# Autodesk Inventor assembly: MG-Encoderplatine
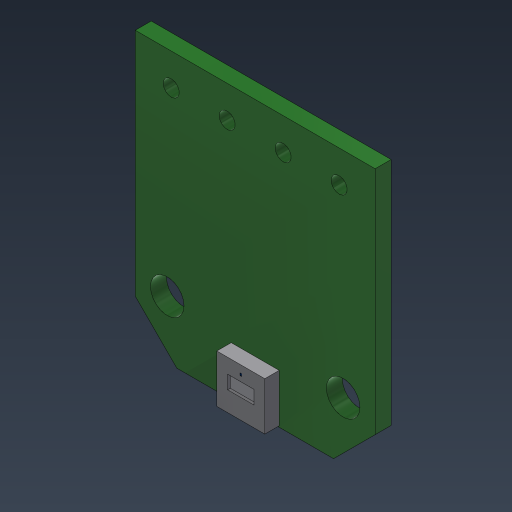
[picture p0: Inventor's stored thumbnail of the model, 512x512]
Saved by Autodesk Inventor 2023.1 (Build 271208000, 208)
## iProperties
Part Number: MG-Encoderplatine
Material: Generisch
Document SubType Name: Assembly
Designer: rYan
Mass: 0.362061 g
Surface Area: 6.73753 cm^2
Volume: 0.271556 cm^3
Density: 1.33328 g/cm^3
Author: rYan
## Documents named in this file (3)
- D:\TIGERsGIT\Hardware\mechanik\2024\Inventor\Robot\Drive Train\Common\MG-Encoderplatine.iam
- D:\TIGERsGIT\Hardware\mechanik\2024\Inventor\Robot\Drive Train\Common\Encoderplatine.ipt
- D:\TIGERsGIT\Hardware\mechanik\2024\Inventor\Purchased Parts\iC-PX Series Encoder.ipt
## Components (2 placed, 2 different names)
1. Encoderplatine:1 — Passend:2, Fluchtend:3, Fluchtend:4
2. iC-PX Series Encoder:1 — Passend:2, Fluchtend:3, Fluchtend:4
## Relationships (3: Flush 2, Mate 1)
- Passend:2 [Mate]: Encoderplatine:1 ↔ iC-PX Series Encoder:1
- Fluchtend:3 [Flush]: Encoderplatine:1 ↔ iC-PX Series Encoder:1
- Fluchtend:4 [Flush] (-1.581 mm): Encoderplatine:1 ↔ iC-PX Series Encoder:1
